# Autodesk Inventor assembly: Counter
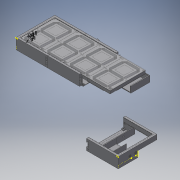
[picture p0: Inventor's stored thumbnail of the model, 180x180]
Saved by Autodesk Inventor 2016 SP2 (Build 200236200, 236)
## iProperties
Created: 2018-06-10
Part Number: Counter
Material: Generisch
Document SubType Name: Assembly
Designer: Nils
Author: Nils
## Documents named in this file (14)
- C:\Users\Nils\Documents\Inventor\Bastelleien\Counter\Counter.iam
- C:\Users\Nils\Documents\Inventor\Bastelleien\Counter\Segment_V4.ipt
- C:\Users\Nils\Documents\Inventor\Bastelleien\Counter\Cover_V2.ipt
- C:\Users\Nils\Documents\Inventor\Bastelleien\Counter\Backplate_V2.ipt
- C:\Users\Nils\Documents\Inventor\Bastelleien\Counter\Bauteil1.ipt
- C:\Users\Nils\Documents\Inventor\Bastelleien\Counter\Bauteil3.ipt
- C:\Users\Nils\Documents\Inventor\Bastelleien\Counter\TopFrame.ipt
- C:\Users\Nils\Documents\Inventor\Bastelleien\Counter\Bauteil1_MIR.ipt
- C:\Users\Nils\Documents\Inventor\Bastelleien\Counter\Scheibe.ipt
- C:\Users\Nils\Documents\Inventor\Bastelleien\Counter\Backplate-housing.ipt
- C:\Users\Nils\Documents\Inventor\Bastelleien\Counter\BatCap.ipt
- C:\Users\Nils\Documents\Inventor\Bastelleien\Counter\BatCap_MIR.ipt
- C:\Users\Nils\Documents\Inventor\Bastelleien\Counter\Zwischenplatt.ipt
- C:\Users\Nils\Documents\Inventor\Bastelleien\Counter\Knopf.ipt
## Components (22 placed, 13 different names)
1. Segment_V4:1 — Passend:3, Passend:4, Fluchtend:1, Fluchtend:2, Fluchtend:3, Passend:11, Fluchtend:4, Fluchtend:5, Fluchtend:6, Fluchtend:26, Fluchtend:27
2. Cover_V2:1 — Passend:3, Fluchtend:7, Fluchtend:8, Fluchtend:9, Passend:14, Fluchtend:10, Fluchtend:11, Fluchtend:12, Passend:21
3. Backplate_V2:1 — Passend:4, Passend:17, Fluchtend:13, Fluchtend:16, Fluchtend:17, Fluchtend:18
4. Segment_V4:2 — Fluchtend:1, Passend:11, Passend:12, Fluchtend:4
5. Cover_V2:2 — Fluchtend:7, Passend:14, Passend:15, Fluchtend:10
6. Backplate_V2:2 — Passend:17, Passend:18, Fluchtend:13, Fluchtend:14, Fluchtend:16
7. Segment_V4:3 — Fluchtend:2, Passend:12, Passend:13, Fluchtend:5
8. Cover_V2:3 — Fluchtend:8, Passend:15, Passend:16, Fluchtend:11
9. Backplate_V2:3 — Passend:18, Passend:19, Fluchtend:14, Fluchtend:15, Fluchtend:17
10. Segment_V4:4 — Fluchtend:3, Passend:13, Fluchtend:6
11. Cover_V2:4 — Fluchtend:9, Passend:16, Fluchtend:12
12. Backplate_V2:4 — Passend:19, Fluchtend:15, Fluchtend:18
13. Scheibe:1 — Fluchtend:26, Fluchtend:27, Passend:21
14. Bauteil1:1 — Fluchtend:21, Fluchtend:22, Fluchtend:31
15. Bauteil3:1
16. TopFrame:1 — Fluchtend:21, Fluchtend:22
17. Backplate-housing:1
18. BatCap:1
19. BatCap_MIR:1
20. Zwischenplatt:1 — Fluchtend:31
21. Knopf:1
22. Bauteil1_MIR:1
## Relationships (41: Flush 23, Mate 18)
- Passend:3 [Mate] (66.118 mm): Segment_V4:1 ↔ Cover_V2:1
- Passend:4 [Mate] (88.205 mm): Segment_V4:1 ↔ Backplate_V2:1
- [Mate] (66.118 mm): Segment_V4:2 ↔ Cover_V2:2
- [Mate] (88.205 mm): Segment_V4:2 ↔ Backplate_V2:2
- [Mate] (66.118 mm): Segment_V4:3 ↔ Cover_V2:3
- [Mate] (88.205 mm): Segment_V4:3 ↔ Backplate_V2:3
- [Mate] (66.118 mm): Segment_V4:4 ↔ Cover_V2:4
- [Mate] (88.205 mm): Segment_V4:4 ↔ Backplate_V2:4
- Fluchtend:1 [Flush]: Segment_V4:1 ↔ Segment_V4:2
- Fluchtend:2 [Flush]: Segment_V4:1 ↔ Segment_V4:3
- Fluchtend:3 [Flush]: Segment_V4:1 ↔ Segment_V4:4
- Passend:11 [Mate]: Segment_V4:1 ↔ Segment_V4:2
- Passend:12 [Mate]: Segment_V4:2 ↔ Segment_V4:3
- Passend:13 [Mate]: Segment_V4:3 ↔ Segment_V4:4
- Fluchtend:4 [Flush]: Segment_V4:1 ↔ Segment_V4:2
- Fluchtend:5 [Flush]: Segment_V4:1 ↔ Segment_V4:3
- Fluchtend:6 [Flush]: Segment_V4:1 ↔ Segment_V4:4
- Fluchtend:7 [Flush]: Cover_V2:1 ↔ Cover_V2:2
- Fluchtend:8 [Flush]: Cover_V2:1 ↔ Cover_V2:3
- Fluchtend:9 [Flush]: Cover_V2:1 ↔ Cover_V2:4
- Passend:14 [Mate]: Cover_V2:1 ↔ Cover_V2:2
- Passend:15 [Mate]: Cover_V2:2 ↔ Cover_V2:3
- Passend:16 [Mate]: Cover_V2:3 ↔ Cover_V2:4
- Fluchtend:10 [Flush]: Cover_V2:1 ↔ Cover_V2:2
- Fluchtend:11 [Flush]: Cover_V2:1 ↔ Cover_V2:3
- Fluchtend:12 [Flush]: Cover_V2:1 ↔ Cover_V2:4
- Passend:17 [Mate]: Backplate_V2:1 ↔ Backplate_V2:2
- Passend:18 [Mate]: Backplate_V2:2 ↔ Backplate_V2:3
- Passend:19 [Mate]: Backplate_V2:3 ↔ Backplate_V2:4
- Fluchtend:13 [Flush]: Backplate_V2:1 ↔ Backplate_V2:2
- Fluchtend:14 [Flush]: Backplate_V2:2 ↔ Backplate_V2:3
- Fluchtend:15 [Flush]: Backplate_V2:3 ↔ Backplate_V2:4
- Fluchtend:16 [Flush]: Backplate_V2:1 ↔ Backplate_V2:2
- Fluchtend:17 [Flush]: Backplate_V2:1 ↔ Backplate_V2:3
- Fluchtend:18 [Flush]: Backplate_V2:1 ↔ Backplate_V2:4
- Fluchtend:21 [Flush]: Bauteil1:1 ↔ TopFrame:1
- Fluchtend:22 [Flush]: Bauteil1:1 ↔ TopFrame:1
- Fluchtend:26 [Flush] (0.75 mm): Segment_V4:1 ↔ Scheibe:1
- Fluchtend:27 [Flush] (0.171 mm): Segment_V4:1 ↔ Scheibe:1
- Passend:21 [Mate] (15.632 mm): Cover_V2:1 ↔ Scheibe:1
- Fluchtend:31 [Flush]: Bauteil1:1 ↔ Zwischenplatt:1
## Named parameters: d18_d12 = 66.118 mm, d19_d13 = 50 mm, d20_d14 = 0 mm, d21_d15 = 88.205 mm, d22_d16 = 50 mm, d23_d17 = 0 mm, d24_d12 = 66.118 mm, d25_d13 = 50 mm, d26_d14 = 0 mm, d27_d15 = 88.205 mm, d28_d16 = 50 mm, d29_d17 = 0 mm, d30_d12 = 66.118 mm, d31_d13 = 50 mm, d32_d14 = 0 mm, d33_d15 = 88.205 mm, d34_d16 = 50 mm, d35_d17 = 0 mm
